# Autodesk Inventor assembly: 100mm omuniwheel
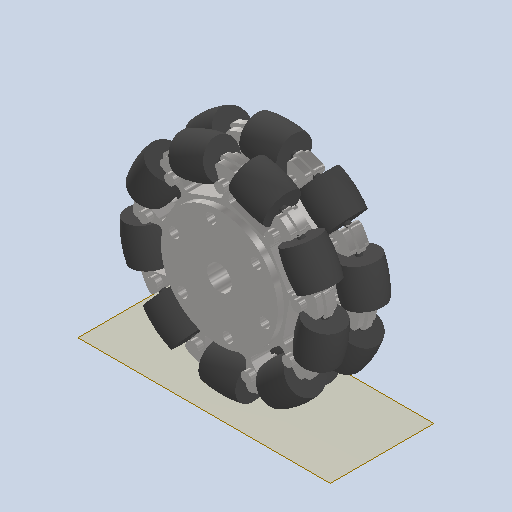
[picture p0: Inventor's stored thumbnail of the model, 512x512]
Saved by Autodesk Inventor 2025.1 (Build 291241000, 241)
## iProperties
Created: 2023-11-21
Part Number: 100mm omuniwheel
Document SubType Name: Assembly
Designer: fhbdh
Author: fhbdh
## Documents named in this file (6)
- C:\Users\haruy\Documents\ロボコン\NHK2025\cad\nagahisa\base_weel\takagi_weel\Workspaces\作業スペース\takagi\omuni_wheel_ver3.0\parts\frequently used parts\タイヤ\omni wheel\100mm wheel\100mm omuniwheel.iam
- C:\Users\haruy\Documents\ロボコン\NHK2025\cad\nagahisa\base_weel\takagi_weel\Workspaces\作業スペース\takagi\omuni_wheel_ver2.0\parts\frequently used parts\タイヤ\omni wheel\100mm wheel\omuni_flame.ipt
- C:\Users\haruy\Documents\ロボコン\NHK2025\cad\nagahisa\base_weel\takagi_weel\Workspaces\作業スペース\takagi\omuni_wheel_ver2.0\parts\frequently used parts\タイヤ\omni wheel\100mm wheel\omuni_rubber.ipt
- C:\Users\haruy\Documents\ロボコン\NHK2025\cad\nagahisa\base_weel\takagi_weel\Workspaces\作業スペース\takagi\omuni_wheel_ver2.0\parts\frequently used parts\タイヤ\omni wheel\100mm wheel\frange.ipt
- C:\Users\haruy\Documents\ロボコン\NHK2025\cad\nagahisa\base_weel\takagi_weel\Workspaces\作業スペース\takagi\omuni_wheel_ver2.0\parts\frequently used parts\タイヤ\omni wheel\100mm wheel\al_shaft.ipt
- C:\Users\haruy\Documents\ロボコン\NHK2025\cad\nagahisa\base_weel\takagi_weel\Workspaces\作業スペース\takagi\omuni_wheel_ver2.0\parts\frequently used parts\タイヤ\omni wheel\100mm wheel\nut.ipt
## Components (27 placed, 5 different names)
1. omuni_flame:1 — 挿入:1, 挿入:2, 挿入:3, 挿入:4, 挿入:5, 挿入:6, 挿入:7, 挿入:8, 挿入:9, 挿入:19, メイト:1, 挿入:20, 挿入:21, 挿入:22
2. omuni_rubber:1 — 挿入:3
3. omuni_rubber:2 — 挿入:4
4. omuni_rubber:3 — 挿入:5
5. omuni_rubber:4 — 挿入:9
6. omuni_rubber:5 — 挿入:8
7. omuni_rubber:6 — 挿入:7
8. omuni_rubber:7 — 挿入:2
9. omuni_rubber:8 — 挿入:6
10. omuni_rubber:9 — 挿入:1, メイト:3
11. frange:1 — 挿入:19, メイト:1
12. omuni_flame:2 — 挿入:28, 挿入:29, 挿入:30, 挿入:31, 挿入:32, メイト:2
13. omuni_rubber:10
14. omuni_rubber:11
15. omuni_rubber:12
16. omuni_rubber:13
17. omuni_rubber:14
18. omuni_rubber:15
19. omuni_rubber:16
20. omuni_rubber:17
21. omuni_rubber:18 — 正接:1
22. al_shaft:1 — 挿入:22, 挿入:28
23. al_shaft:2 — 挿入:21, 挿入:29
24. al_shaft:3 — 挿入:20
25. nut:1 — 挿入:32
26. nut:2 — 挿入:30
27. nut:3 — 挿入:31
## Relationships (31: Insert 27, Mate 3, Tangent 1)
- 挿入:1 [Insert]: omuni_flame:1 ↔ omuni_rubber:9
- 挿入:2 [Insert]: omuni_flame:1 ↔ omuni_rubber:7
- 挿入:3 [Insert]: omuni_flame:1 ↔ omuni_rubber:1
- 挿入:4 [Insert]: omuni_flame:1 ↔ omuni_rubber:2
- 挿入:5 [Insert]: omuni_flame:1 ↔ omuni_rubber:3
- 挿入:6 [Insert]: omuni_flame:1 ↔ omuni_rubber:8
- 挿入:7 [Insert]: omuni_flame:1 ↔ omuni_rubber:6
- 挿入:8 [Insert]: omuni_flame:1 ↔ omuni_rubber:5
- 挿入:9 [Insert]: omuni_flame:1 ↔ omuni_rubber:4
- [Insert]: omuni_flame:2 ↔ omuni_rubber:18
- [Insert]: omuni_flame:2 ↔ omuni_rubber:16
- [Insert]: omuni_flame:2 ↔ omuni_rubber:10
- [Insert]: omuni_flame:2 ↔ omuni_rubber:11
- [Insert]: omuni_flame:2 ↔ omuni_rubber:12
- [Insert]: omuni_flame:2 ↔ omuni_rubber:17
- [Insert]: omuni_flame:2 ↔ omuni_rubber:15
- [Insert]: omuni_flame:2 ↔ omuni_rubber:14
- [Insert]: omuni_flame:2 ↔ omuni_rubber:13
- 挿入:19 [Insert]: omuni_flame:1 ↔ frange:1
- メイト:1 [Mate]: omuni_flame:1 ↔ frange:1
- 挿入:20 [Insert]: omuni_flame:1 ↔ al_shaft:3
- 挿入:21 [Insert]: omuni_flame:1 ↔ al_shaft:2
- 挿入:22 [Insert]: omuni_flame:1 ↔ al_shaft:1
- 挿入:28 [Insert]: omuni_flame:2 ↔ al_shaft:1
- 挿入:29 [Insert]: omuni_flame:2 ↔ al_shaft:2
- 挿入:30 [Insert]: omuni_flame:2 ↔ nut:2
- 挿入:31 [Insert]: omuni_flame:2 ↔ nut:3
- 挿入:32 [Insert]: omuni_flame:2 ↔ nut:1
- 正接:1 [Tangent]: omuni_rubber:18
- メイト:2 [Mate]: omuni_flame:2
- メイト:3 [Mate]: omuni_rubber:9
## Named parameters: d11_d0 = 0 mm, d12_d1 = 0 mm, d13_d2 = 0 mm, d14_d3 = 0 mm, d15_d4 = 0 mm, d16_d5 = 0 mm, d17_d6 = 0 mm, d18_d7 = 0 mm, d19_d8 = 0 mm
